# Autodesk Inventor assembly: TABLE
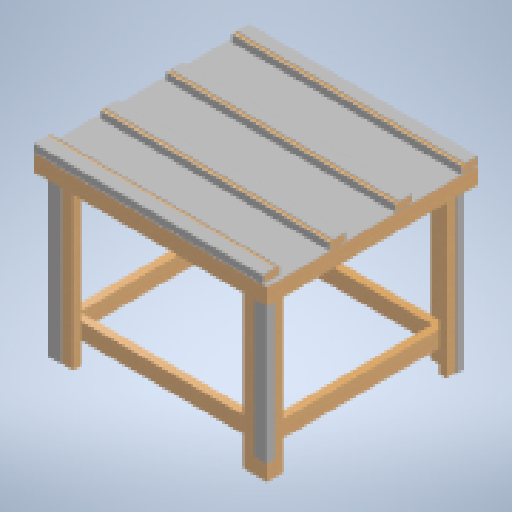
[picture p0: Inventor's stored thumbnail of the model, 512x512]
Saved by Autodesk Inventor 2023 (Build 270158000, 158)
## iProperties
Created: 2022-07-13
Part Number: TABLE
Document SubType Name: Assembly
Designer: plebbb
Author: plebbb
## Documents named in this file (6)
- D:\Users\plebbb\Desktop\CNC_Project\TABLE.iam
- D:\Users\plebbb\Desktop\CNC_Project\Wood_X_Frame.iam
- D:\Users\plebbb\Desktop\CNC_Project\Flat_plate.ipt
- D:\Users\plebbb\Desktop\CNC_Project\WOODLEG.iam
- D:\Users\plebbb\Desktop\CNC_Project\WOOD\FRAMEBOX.iam
- D:\Users\plebbb\Desktop\CNC_Project\FrameBoxLow.iam
## Components (11 placed, 5 different names)
1. Wood_X_Frame:1 [sub-assembly]
2. Flat_plate:1
3. WOODLEG:1 [sub-assembly]
4. WOODLEG:2 [sub-assembly]
5. WOODLEG:3 [sub-assembly]
6. WOODLEG:4 [sub-assembly]
7. FRAMEBOX:1 [sub-assembly]
8. FrameBoxLow:1 [sub-assembly]
9. Wood_X_Frame:2 [sub-assembly]
10. Wood_X_Frame:3 [sub-assembly]
11. Wood_X_Frame:4 [sub-assembly]
## Component patterns: (3 elements, first: Wood_X_Frame:2)
## Relationships (33: Mate 22, Flush 11)
- [Flush]: Flat_plate:1 ↔ Wood_X_Frame:2
- [Flush]: Flat_plate:1 ↔ Wood_X_Frame:2
- [Flush]: Flat_plate:1 ↔ Wood_X_Frame:2
- [Mate]: Flat_plate:1 ↔ FRAMEBOX:1
- [Flush]: Flat_plate:1 ↔ FRAMEBOX:1
- [Flush]: Flat_plate:1 ↔ FRAMEBOX:1
- [Mate]: Flat_plate:1 ↔ FRAMEBOX:1
- [Flush]: Flat_plate:1 ↔ FRAMEBOX:1
- [Flush]: Flat_plate:1 ↔ FRAMEBOX:1
- [Mate]: Flat_plate:1 ↔ FRAMEBOX:1
- [Mate]: Flat_plate:1 ↔ FRAMEBOX:1
- [Mate]: WOODLEG:1 ↔ FRAMEBOX:1
- [Mate]: Flat_plate:1 ↔ WOODLEG:1
- [Mate]: WOODLEG:1 ↔ FRAMEBOX:1
- [Mate]: WOODLEG:1 ↔ FRAMEBOX:1
- [Mate]: Flat_plate:1 ↔ WOODLEG:2
- [Mate]: WOODLEG:2 ↔ FRAMEBOX:1
- [Mate]: WOODLEG:2 ↔ FRAMEBOX:1
- [Mate]: WOODLEG:4 ↔ FRAMEBOX:1
- [Mate]: Flat_plate:1 ↔ WOODLEG:4
- [Mate]: WOODLEG:4 ↔ FRAMEBOX:1
- [Mate]: WOODLEG:3 ↔ FRAMEBOX:1
- [Mate]: WOODLEG:3 ↔ FRAMEBOX:1
- [Flush]: WOODLEG:1 ↔ WOODLEG:3
- [Flush]: WOODLEG:1 ↔ WOODLEG:2
- [Flush]: WOODLEG:2 ↔ WOODLEG:4
- [Mate]: WOODLEG:4 ↔ FrameBoxLow:1
- [Mate]: WOODLEG:3 ↔ FrameBoxLow:1
- [Mate]: WOODLEG:1 ↔ FrameBoxLow:1
- [Mate]: WOODLEG:2 ↔ FrameBoxLow:1
- [Mate]: WOODLEG:2 ↔ FrameBoxLow:1
- [Mate]: WOODLEG:3 ↔ FrameBoxLow:1
- [Flush] (127 mm): WOODLEG:1 ↔ FrameBoxLow:1
